# Autodesk Inventor assembly: Enclosure Assembly
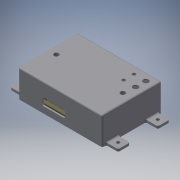
[picture p0: Inventor's stored thumbnail of the model, 180x180]
Saved by Autodesk Inventor 2019 (Build 230136000, 136)
## iProperties
Created: 2022-03-18
Part Number: Enclosure Assembly
Document SubType Name: Assembly
Designer: Lix
Author: Lix
## Documents named in this file (3)
- G:\Project\Hybrids\HexaWall\Inventor\pcb\Enclosure Assembly.iam
- G:\Project\Hybrids\HexaWall\Inventor\pcb\Enclosure v1.ipt
- G:\Project\Hybrids\HexaWall\Inventor\pcb\HexaWall-v1.1 v7.iam
## Components (2 placed, 2 different names)
1. Enclosure v1:1 — Mate:3, Mate:4, Mate:5
2. HexaWall-v1.1 v7:1 [sub-assembly] — Mate:3, Mate:4, Mate:5
## Relationships (3: Mate 3)
- Mate:3: Enclosure v1:1 ↔ HexaWall-v1.1 v7:1
- Mate:4: Enclosure v1:1 ↔ HexaWall-v1.1 v7:1
- Mate:5: Enclosure v1:1 ↔ HexaWall-v1.1 v7:1
